# Autodesk Inventor assembly: stand
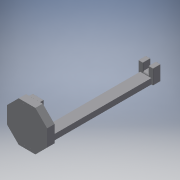
[picture p0: Inventor's stored thumbnail of the model, 180x180]
Saved by Autodesk Inventor 2019 (Build 230136000, 136)
## iProperties
Created: 2019-12-27
Part Number: stand
Material: Типовые
Document SubType Name: Assembly
Designer: stepa
Author: stepa
## Documents named in this file (5)
- C:\Users\stepa\Documents\Inventor\Shamisen\stand.iam
- C:\Users\stepa\Documents\Inventor\Shamisen\stand_bottom.ipt
- C:\Users\stepa\Documents\Inventor\Shamisen\stand_stop.ipt
- C:\Users\stepa\Documents\Inventor\Shamisen\stand_vert.ipt
- C:\Users\stepa\Documents\Inventor\Shamisen\stand_holder.ipt
## Components (4 placed, 4 different names)
1. stand_bottom:1 — Совмещение:1, Совмещение:2, Совмещение:3, Совмещение:4, Заподлицо:1, Совмещение:7
2. stand_stop:1 — Совмещение:1, Совмещение:2, Совмещение:3
3. stand_vert:1 — Совмещение:4, Заподлицо:1, Совмещение:5, Совмещение:6, Заподлицо:2, Совмещение:7
4. stand_holder:1 — Совмещение:5, Совмещение:6, Заподлицо:2
## Relationships (9: Mate 7, Flush 2)
- Совмещение:1 [Mate]: stand_bottom:1 ↔ stand_stop:1
- Совмещение:2 [Mate]: stand_bottom:1 ↔ stand_stop:1
- Совмещение:3 [Mate]: stand_bottom:1 ↔ stand_stop:1
- Совмещение:4 [Mate]: stand_bottom:1 ↔ stand_vert:1
- Заподлицо:1 [Flush]: stand_bottom:1 ↔ stand_vert:1
- Совмещение:5 [Mate]: stand_vert:1 ↔ stand_holder:1
- Совмещение:6 [Mate]: stand_vert:1 ↔ stand_holder:1
- Заподлицо:2 [Flush]: stand_vert:1 ↔ stand_holder:1
- Совмещение:7 [Mate]: stand_bottom:1 ↔ stand_vert:1
